# Autodesk Inventor assembly: Chassis Assembly
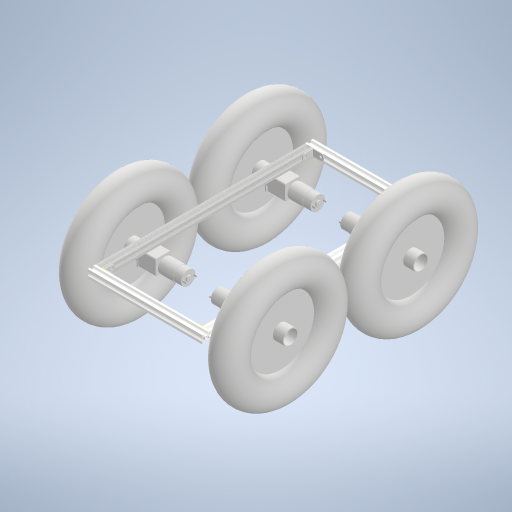
[picture p0: Inventor's stored thumbnail of the model, 512x512]
Saved by Autodesk Inventor 2024 (Build 280153000, 153)
## iProperties
Created: 2023-10-09
Part Number: Chassis Assembly
Document SubType Name: Assembly
Designer: luke.macenski3281
Author: luke.macenski3281
## Documents named in this file (7)
- C:\Users\luke.macenski3281\OneDrive - Butler Technology and Career Development Schools\Desktop\12.11.23\Chassis Assembly.iam
- C:\Users\luke.macenski3281\OneDrive - Butler Technology and Career Development Schools\Desktop\12.11.23\20mm_V-Rail_Extrusion Long.ipt
- C:\Users\luke.macenski3281\OneDrive - Butler Technology and Career Development Schools\Desktop\12.11.23\20mm_V-Rail_Extrusion Short.ipt
- C:\Users\luke.macenski3281\OneDrive - Butler Technology and Career Development Schools\Desktop\12.11.23\Right Angle.ipt
- C:\Users\luke.macenski3281\OneDrive - Butler Technology and Career Development Schools\Desktop\12.11.23\DC Motor.ipt
- C:\Users\luke.macenski3281\OneDrive - Butler Technology and Career Development Schools\Desktop\12.11.23\Savior Wheel.ipt
- C:\Users\luke.macenski3281\OneDrive - Butler Technology and Career Development Schools\Desktop\12.11.23\Wheel Washer.ipt
## Components (20 placed, 6 different names)
1. 20mm_V-Rail_Extrusion Long:1 — Mate:2, Flush:3, Flush:4, Flush:5, Flush:6, Mate:8, Mate:9, Flush:11, Flush:12, Mate:15, Mate:16
2. 20mm_V-Rail_Extrusion Short:1 — Mate:4, Flush:5, Flush:6, Mate:10, Flush:9, Mate:12, Flush:16, Flush:17
3. 20mm_V-Rail_Extrusion Long:2 — Mate:1, Mate:3, Flush:1, Flush:2, Mate:4, Mate:5, Flush:7, Mate:11, Flush:10, Flush:13, Flush:14, Mate:13, Mate:14
4. 20mm_V-Rail_Extrusion Short:2 — Mate:1, Mate:2, Mate:3, Flush:1, Flush:2, Flush:3, Flush:4, Mate:6, Mate:7, Flush:8, Mate:17, Flush:15
5. Right Angle:1 — Mate:7, Mate:8, Flush:8
6. Right Angle:2 — Mate:5, Mate:6, Flush:7
7. Right Angle:3 — Mate:9, Mate:10, Flush:9
8. Right Angle:4 — Mate:11, Mate:12, Flush:10
9. DC Motor:1 — Flush:11, Mate:15, Flush:17, Insert:3
10. DC Motor:2 — Flush:14, Mate:14, Mate:17, Insert:2
11. DC Motor:3 — Flush:12, Mate:16, Flush:15, Insert:4
12. DC Motor:4 — Flush:13, Mate:13, Flush:16, Insert:1
13. Savior Wheel:1 — Insert:5
14. Savior Wheel:2 — Insert:6
15. Savior Wheel:3 — Insert:8
16. Savior Wheel:4 — Insert:7
17. Wheel Washer:2 — Insert:2, Insert:5
18. Wheel Washer:1 — Insert:4, Insert:7
19. Wheel Washer:3 — Insert:1, Insert:6
20. Wheel Washer:4 — Insert:3, Insert:8
## Relationships (42: Mate 17, Flush 17, Insert 8)
- Mate:1: 20mm_V-Rail_Extrusion Long:2 ↔ 20mm_V-Rail_Extrusion Short:2
- Mate:2: 20mm_V-Rail_Extrusion Long:1 ↔ 20mm_V-Rail_Extrusion Short:2
- Mate:3: 20mm_V-Rail_Extrusion Long:2 ↔ 20mm_V-Rail_Extrusion Short:2
- Flush:1: 20mm_V-Rail_Extrusion Long:2 ↔ 20mm_V-Rail_Extrusion Short:2
- Flush:2: 20mm_V-Rail_Extrusion Long:2 ↔ 20mm_V-Rail_Extrusion Short:2
- Flush:3: 20mm_V-Rail_Extrusion Long:1 ↔ 20mm_V-Rail_Extrusion Short:2
- Flush:4: 20mm_V-Rail_Extrusion Long:1 ↔ 20mm_V-Rail_Extrusion Short:2
- Mate:4: 20mm_V-Rail_Extrusion Short:1 ↔ 20mm_V-Rail_Extrusion Long:2
- Flush:5: 20mm_V-Rail_Extrusion Long:1 ↔ 20mm_V-Rail_Extrusion Short:1
- Flush:6: 20mm_V-Rail_Extrusion Long:1 ↔ 20mm_V-Rail_Extrusion Short:1
- Mate:5: 20mm_V-Rail_Extrusion Long:2 ↔ Right Angle:2
- Mate:6: 20mm_V-Rail_Extrusion Short:2 ↔ Right Angle:2
- Flush:7: 20mm_V-Rail_Extrusion Long:2 ↔ Right Angle:2
- Mate:7: 20mm_V-Rail_Extrusion Short:2 ↔ Right Angle:1
- Mate:8: 20mm_V-Rail_Extrusion Long:1 ↔ Right Angle:1
- Flush:8: 20mm_V-Rail_Extrusion Short:2 ↔ Right Angle:1
- Mate:9: 20mm_V-Rail_Extrusion Long:1 ↔ Right Angle:3
- Mate:10: 20mm_V-Rail_Extrusion Short:1 ↔ Right Angle:3
- Flush:9: 20mm_V-Rail_Extrusion Short:1 ↔ Right Angle:3
- Mate:11: 20mm_V-Rail_Extrusion Long:2 ↔ Right Angle:4
- Mate:12: 20mm_V-Rail_Extrusion Short:1 ↔ Right Angle:4
- Flush:10: 20mm_V-Rail_Extrusion Long:2 ↔ Right Angle:4
- Flush:11: 20mm_V-Rail_Extrusion Long:1 ↔ DC Motor:1
- Flush:12: 20mm_V-Rail_Extrusion Long:1 ↔ DC Motor:3
- Flush:13: 20mm_V-Rail_Extrusion Long:2 ↔ DC Motor:4
- Flush:14: 20mm_V-Rail_Extrusion Long:2 ↔ DC Motor:2
- Mate:13: 20mm_V-Rail_Extrusion Long:2 ↔ DC Motor:4
- Mate:14: 20mm_V-Rail_Extrusion Long:2 ↔ DC Motor:2
- Mate:15: 20mm_V-Rail_Extrusion Long:1 ↔ DC Motor:1
- Mate:16: 20mm_V-Rail_Extrusion Long:1 ↔ DC Motor:3
- Mate:17 (127 mm): 20mm_V-Rail_Extrusion Short:2 ↔ DC Motor:2
- Flush:15 (127 mm): 20mm_V-Rail_Extrusion Short:2 ↔ DC Motor:3
- Flush:16 (76.2 mm): 20mm_V-Rail_Extrusion Short:1 ↔ DC Motor:4
- Flush:17 (76.2 mm): 20mm_V-Rail_Extrusion Short:1 ↔ DC Motor:1
- Insert:1 (19.05 mm): DC Motor:4 ↔ Wheel Washer:3
- Insert:2 (17.78 mm): DC Motor:2 ↔ Wheel Washer:2
- Insert:3 (19.05 mm): DC Motor:1 ↔ Wheel Washer:4
- Insert:4 (-19.05 mm): DC Motor:3 ↔ Wheel Washer:1
- Insert:5 (-20.32 mm): Savior Wheel:1 ↔ Wheel Washer:2
- Insert:6 (20.32 mm): Savior Wheel:2 ↔ Wheel Washer:3
- Insert:7 (20.32 mm): Savior Wheel:4 ↔ Wheel Washer:1
- Insert:8 (-63.5 mm): Savior Wheel:3 ↔ Wheel Washer:4
